# Autodesk Inventor assembly: Foerderband_150cm
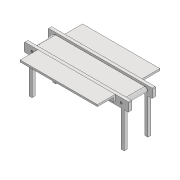
[picture p0: Inventor's stored thumbnail of the model, 180x180]
Saved by Autodesk Inventor 2020 (Build 240168000, 168)
## iProperties
Created: 2020-03-18
Part Number: Foerderband_150cm
Document SubType Name: Assembly
Designer: franz
Author: franz
## Documents named in this file (6)
- E:\Privat\Projekte\SPS_Training\Unity_SPS_Simulation\Unity_SPS_Schrittkette\CAD\Foerderband_V1\Foerderband_150cm\Foerderband_150cm.iam
- E:\Privat\Projekte\SPS_Training\Unity_SPS_Simulation\Unity_SPS_Schrittkette\CAD\Foerderband_V1\Foerderband_150cm\Gestell_Seite.ipt
- E:\Privat\Projekte\SPS_Training\Unity_SPS_Simulation\Unity_SPS_Schrittkette\CAD\Foerderband_V1\Foerderband_150cm\Gestell_Seite_MIR.ipt
- E:\Privat\Projekte\SPS_Training\Unity_SPS_Simulation\Unity_SPS_Schrittkette\CAD\Foerderband_V1\Foerderband_150cm\Foerderbandrollen.ipt
- E:\Privat\Projekte\SPS_Training\Unity_SPS_Simulation\Unity_SPS_Schrittkette\CAD\Foerderband_V1\Foerderband_150cm\Band.ipt
- E:\Privat\Projekte\SPS_Training\Unity_SPS_Simulation\Unity_SPS_Schrittkette\CAD\Foerderband_V1\Foerderband_150cm\Seitboard.ipt
## Components (7 placed, 5 different names)
1. Gestell_Seite:1 — Drehbar:1, Drehbar:2, Starr:1
2. Gestell_Seite_MIR:1 — Drehbar:3, Drehbar:4, Passend:3, Starr:2
3. Foerderbandrollen:1 — Drehbar:2, Drehbar:4, Passend:2
4. Foerderbandrollen:2 — Drehbar:1, Drehbar:3, Passend:1
5. Band:1 — Passend:1, Passend:2, Passend:3
6. Seitboard:1 — Starr:1
7. Seitboard:2 — Starr:2
## Relationships (9: RevoluteJoint 4, Mate 3, WeldJoint 2)
- Drehbar:1 [RevoluteJoint]: Gestell_Seite:1 ↔ Foerderbandrollen:2
- Drehbar:2 [RevoluteJoint]: Gestell_Seite:1 ↔ Foerderbandrollen:1
- Drehbar:3 [RevoluteJoint]: Gestell_Seite_MIR:1 ↔ Foerderbandrollen:2
- Drehbar:4 [RevoluteJoint]: Gestell_Seite_MIR:1 ↔ Foerderbandrollen:1
- Passend:1 [Mate]: Foerderbandrollen:2 ↔ Band:1
- Passend:2 [Mate]: Foerderbandrollen:1 ↔ Band:1
- Passend:3 [Mate] (5 mm): Gestell_Seite_MIR:1 ↔ Band:1
- Starr:1 [WeldJoint]: Gestell_Seite:1 ↔ Seitboard:1
- Starr:2 [WeldJoint]: Gestell_Seite_MIR:1 ↔ Seitboard:2
